# Autodesk Inventor assembly: V4SlapperTower
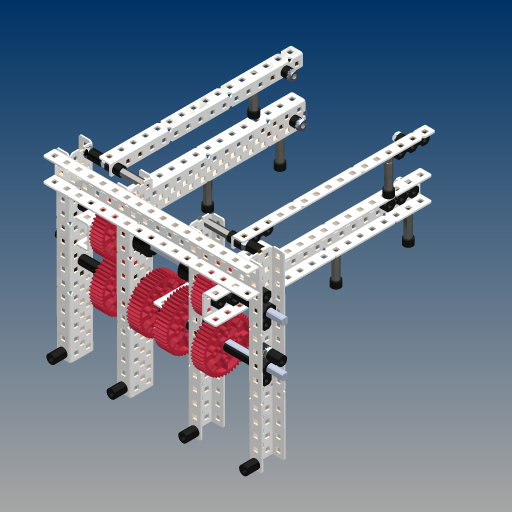
[picture p0: Inventor's stored thumbnail of the model, 512x512]
Saved by Autodesk Inventor 2023 (Build 270158000, 158)
## iProperties
Created: 2024-01-13
Part Number: V4SlapperTower
Document SubType Name: Assembly
Designer: eddie
Author: eddie
## Documents named in this file (30)
- C:\Users\eddie\Documents\81208X-Over-Under-CAD\V4\V4SlapperTower.iam
- C:\Users\eddie\Documents\81208X-Over-Under-CAD\VEX-CAD-Inventor-1.4.0\Structure\C Channel\Aluminum 1x2x1\Alu C 1x2x1x17.ipt
- C:\Users\eddie\Documents\81208X-Over-Under-CAD\VEX-CAD-Inventor-1.4.0\Structure\C Channel\Aluminum 1x2x1\Alu C 1x2x1x15.ipt
- C:\Users\eddie\Documents\81208X-Over-Under-CAD\VEX-CAD-Inventor-1.4.0\Motion\Spacers\Spacer Nylon .375 OD\NSpacer .375 OD x .500.ipt
- C:\Users\eddie\Documents\81208X-Over-Under-CAD\VEX-CAD-Inventor-1.4.0\Motion\Spacers\Spacer Nylon .375 OD.ipt
- C:\Users\eddie\Documents\81208X-Over-Under-CAD\VEX-CAD-Inventor-1.4.0\Motion\Spacers\Spacer Nylon .375 OD\NSpacer .375 OD x .250.ipt
- C:\Users\eddie\Documents\81208X-Over-Under-CAD\VEX-CAD-Inventor-1.4.0\Motion\Shaft HS\HS Bearing Flat.ipt
- C:\Users\eddie\Documents\81208X-Over-Under-CAD\VEX-CAD-Inventor-1.4.0\Motion\Gears\HS Gear\HS 48T Gear, Square.iam
- C:\Users\eddie\Documents\81208X-Over-Under-CAD\VEX-CAD-Inventor-1.4.0\Motion\Gears\HS Gear.iam
- C:\Users\eddie\Documents\81208X-Over-Under-CAD\VEX-CAD-Inventor-1.4.0\Motion\Spacers\Spacer Nylon .375 OD\NSpacer .375 OD x .125.ipt
- C:\Users\eddie\Documents\81208X-Over-Under-CAD\VEX-CAD-Inventor-1.4.0\Structure\Hardware\Nut Keps.ipt
- C:\Users\eddie\Documents\81208X-Over-Under-CAD\VEX-CAD-Inventor-1.4.0\Structure\Standoff\Standoff 1.00.ipt
- C:\Users\eddie\Documents\81208X-Over-Under-CAD\VEX-CAD-Inventor-1.4.0\Structure\Standoff.ipt
- C:\Users\eddie\Documents\81208X-Over-Under-CAD\VEX-CAD-Inventor-1.4.0\Structure\Angle\Aluminum\1x1\Alu Angle 1x1x16.ipt
- C:\Users\eddie\Documents\81208X-Over-Under-CAD\VEX-CAD-Inventor-1.4.0\Motion\Shaft LS\Bearing Flat.ipt
- C:\Users\eddie\Documents\81208X-Over-Under-CAD\VEX-CAD-Inventor-1.4.0\Structure\Hardware\Nut Nylock.ipt
- C:\Users\eddie\Documents\81208X-Over-Under-CAD\VEX-CAD-Inventor-1.4.0\Structure\C Channel\Aluminum 1x2x1\Alu C 1x2x1x18.ipt
- C:\Users\eddie\Documents\81208X-Over-Under-CAD\VEX-CAD-Inventor-1.4.0\Structure\C Channel\Aluminum 1x2x1\Alu C 1x2x1x15_MIR1.ipt
- C:\Users\eddie\Documents\81208X-Over-Under-CAD\VEX-CAD-Inventor-1.4.0\Motion\Shaft HS\HS Bearing Flat_MIR.ipt
- C:\Users\eddie\Documents\81208X-Over-Under-CAD\VEX-CAD-Inventor-1.4.0\Motion\Gears\HS Gear\HS 48T Gear, Square_MIR.iam
- C:\Users\eddie\Documents\81208X-Over-Under-CAD\VEX-CAD-Inventor-1.4.0\Structure\Hardware\Nut Keps_MIR.ipt
- C:\Users\eddie\Documents\81208X-Over-Under-CAD\VEX-CAD-Inventor-1.4.0\Structure\Angle\Aluminum\1x1\Alu Angle 1x1x16_MIR.ipt
- C:\Users\eddie\Documents\81208X-Over-Under-CAD\VEX-CAD-Inventor-1.4.0\Motion\Shaft LS\Bearing Flat_MIR1.ipt
- C:\Users\eddie\Documents\81208X-Over-Under-CAD\VEX-CAD-Inventor-1.4.0\Structure\Hardware\Nut Nylock_MIR.ipt
- C:\Users\eddie\Documents\81208X-Over-Under-CAD\VEX-CAD-Inventor-1.4.0\Structure\C Channel\Aluminum 1x2x1\Alu C 1x2x1x18_MIR.ipt
- C:\Users\eddie\Documents\81208X-Over-Under-CAD\VEX-CAD-Inventor-1.4.0\Structure\C Channel\Aluminum 1x2x1\Alu C 1x2x1x9.ipt
- C:\Users\eddie\Documents\81208X-Over-Under-CAD\VEX-CAD-Inventor-1.4.0\Motion\Shaft HS\Shaft HS\Shaft HS 8.5 in.ipt
- C:\Users\eddie\Documents\81208X-Over-Under-CAD\VEX-CAD-Inventor-1.4.0\Motion\Shaft HS\Shaft HS.ipt
- C:\Users\eddie\Documents\81208X-Over-Under-CAD\VEX-CAD-Inventor-1.4.0\Motion\Shaft HS\HS Shaft Collar.ipt
- C:\Users\eddie\Documents\81208X-Over-Under-CAD\VEX-CAD-Inventor-1.4.0\Structure\Standoff\Standoff .25.ipt
## Components (100 placed, 25 different names)
1. Alu C 1x2x1x15:1 — Insert:8, Insert:9, Insert:24, Insert:25, Insert:36, Insert:75, Insert:76
2. Alu C 1x2x1x15:2 — Insert:7, Insert:13, Insert:17, Insert:28, Insert:31, Insert:74, Insert:77, Insert:84
3. NSpacer .375 OD x .500:1 — Insert:8
4. NSpacer .375 OD x .500:2 — Insert:7
5. NSpacer .375 OD x .500:5 — Insert:9, Insert:11
6. NSpacer .375 OD x .250:7 — Insert:11, Insert:12
7. NSpacer .375 OD x .500:8 — Insert:12
8. HS Bearing Flat:1 — Insert:13, Insert:14
9. NSpacer .375 OD x .250:9 — Insert:14, Insert:15
10. HS 48T Gear, Square:1 [sub-assembly] — Insert:15, Insert:38
11. HS Bearing Flat:2 — Insert:17, Insert:18
12. NSpacer .375 OD x .250:11 — Insert:18, Insert:19
13. HS 48T Gear, Square:2 [sub-assembly] — Insert:19, Insert:20
14. NSpacer .375 OD x .125:12 — Insert:20, Insert:21
15. NSpacer .375 OD x .500:13 — Insert:21, Insert:22
16. NSpacer .375 OD x .500:14 — Insert:22, Insert:23
17. NSpacer .375 OD x .250:15 — Insert:23
18. HS Bearing Flat:3 — Insert:24, Insert:82
19. HS Bearing Flat:4 — Insert:25, Insert:26, Insert:83
20. Nut Keps:1 — Insert:26, Insert:27
21. NSpacer .375 OD x .500:16 — Insert:27
22. NSpacer .375 OD x .250:17 — Insert:28, Insert:29
23. NSpacer .375 OD x .125:18 — Insert:29, Insert:30
24. HS 48T Gear, Square:3 [sub-assembly] — Insert:30
25. Standoff 1.00:1 — Insert:31, Insert:32
26. NSpacer .375 OD x .250:19 — Insert:32, Insert:33
27. Alu Angle 1x1x16:1 — Insert:33, Insert:34, Insert:78, Insert:86, Insert:102, Insert:108
28. Bearing Flat:1 — Insert:34, Insert:35, Insert:78
29. Nut Nylock:1 — Insert:35
30. Nut Keps:2 — Insert:36, Insert:37
31. NSpacer .375 OD x .500:20 — Insert:37
32. Alu C 1x2x1x18:1 — Insert:38, Insert:39, Insert:40, Insert:87, Insert:94, Insert:100, Insert:116
33. HS Bearing Flat:5 — Insert:39, Insert:40
34. Alu C 1x2x1x15_MIR1:1 — Insert:41, Insert:43, Insert:56, Insert:57, Insert:68, Insert:73
35. Alu C 1x2x1x15_MIR1:2 — Insert:42, Insert:46, Insert:49, Insert:60, Insert:63, Insert:85
36. NSpacer .375 OD x .500:21 — Insert:41
37. NSpacer .375 OD x .500:22 — Insert:42
38. NSpacer .375 OD x .500:23 — Insert:43, Insert:44
39. NSpacer .375 OD x .250:24 — Insert:44, Insert:45
40. NSpacer .375 OD x .500:25 — Insert:45
41. HS Bearing Flat_MIR:1 — Insert:46, Insert:47
42. NSpacer .375 OD x .250:26 — Insert:47, Insert:48
43. HS 48T Gear, Square_MIR:1 [sub-assembly] — Insert:48, Insert:70
44. HS Bearing Flat_MIR:2 — Insert:49, Insert:50
45. NSpacer .375 OD x .250:27 — Insert:50, Insert:51
46. HS 48T Gear, Square_MIR:2 [sub-assembly] — Insert:51, Insert:52
47. NSpacer .375 OD x .125:28 — Insert:52, Insert:53
48. NSpacer .375 OD x .500:29 — Insert:53, Insert:54
49. NSpacer .375 OD x .500:30 — Insert:54, Insert:55
50. NSpacer .375 OD x .250:31 — Insert:55
51. HS Bearing Flat_MIR:3 — Insert:56
52. HS Bearing Flat_MIR:4 — Insert:57, Insert:58
53. Nut Keps_MIR:1 — Insert:58, Insert:59
54. NSpacer .375 OD x .500:32 — Insert:59
55. NSpacer .375 OD x .250:33 — Insert:60, Insert:61
56. NSpacer .375 OD x .125:34 — Insert:61, Insert:62
57. HS 48T Gear, Square_MIR:3 [sub-assembly] — Insert:62, Insert:79
58. Standoff 1.00:2 — Insert:63, Insert:64
59. NSpacer .375 OD x .250:35 — Insert:64, Insert:65
60. Alu Angle 1x1x16_MIR:1 — Insert:65, Insert:66, Insert:88, Insert:105, Insert:110
61. Bearing Flat_MIR1:1 — Insert:66, Insert:67
62. Nut Nylock_MIR:1 — Insert:67
63. Nut Keps_MIR:2 — Insert:68, Insert:69
64. NSpacer .375 OD x .500:36 — Insert:69
65. Alu C 1x2x1x18_MIR:1 — Insert:70, Insert:71, Insert:72, Insert:89, Insert:96, Insert:97, Insert:114
66. HS Bearing Flat_MIR:5 — Insert:71, Insert:72
67. Alu C 1x2x1x17:1 — Insert:73, Insert:74, Insert:75, Insert:76, Insert:77
68. Alu C 1x2x1x9:1 — Insert:79, Insert:80
69. NSpacer .375 OD x .500:37 — Insert:80, Insert:81
70. NSpacer .375 OD x .125:38 — Insert:81
71. Shaft HS 8.5 in:1 — Insert:82
72. Shaft HS 8.5 in:2 — Insert:83
73. HS Shaft Collar:1 — Insert:84
74. HS Shaft Collar:2 — Insert:85
75. Bearing Flat:2 — Insert:86
76. Bearing Flat:3 — Insert:87
77. Bearing Flat:4 — Insert:88
78. Bearing Flat:5 — Insert:89
79. Standoff 1.00:5 — Insert:94, Insert:95
80. NSpacer .375 OD x .250:41 — Insert:95
81. Standoff 1.00:6 — Insert:96, Insert:98
82. Standoff 1.00:7 — Insert:97, Insert:99
83. NSpacer .375 OD x .250:42 — Insert:98
84. NSpacer .375 OD x .250:43 — Insert:99
85. Standoff 1.00:8 — Insert:100, Insert:101
86. NSpacer .375 OD x .250:44 — Insert:101
87. Standoff .25:9 — Insert:102, Insert:103
88. Standoff 1.00:10 — Insert:103, Insert:104
89. NSpacer .375 OD x .250:45 — Insert:104
90. Standoff .25:11 — Insert:105, Insert:106
91. Standoff 1.00:12 — Insert:106, Insert:107
92. NSpacer .375 OD x .250:46 — Insert:107
93. NSpacer .375 OD x .250:47 — Insert:108, Insert:109
94. Nut Keps:3 — Insert:109
95. NSpacer .375 OD x .250:48 — Insert:110, Insert:111
96. Nut Keps:4 — Insert:111
97. NSpacer .375 OD x .250:50 — Insert:114, Insert:115
98. Nut Keps:6 — Insert:115
99. NSpacer .375 OD x .250:51 — Insert:116, Insert:117
100. Nut Keps:7 — Insert:117
## Relationships (103: Insert 103)
- Insert:7: Alu C 1x2x1x15:2 ↔ NSpacer .375 OD x .500:2
- Insert:8: Alu C 1x2x1x15:1 ↔ NSpacer .375 OD x .500:1
- Insert:9: Alu C 1x2x1x15:1 ↔ NSpacer .375 OD x .500:5
- Insert:11: NSpacer .375 OD x .500:5 ↔ NSpacer .375 OD x .250:7
- Insert:12: NSpacer .375 OD x .250:7 ↔ NSpacer .375 OD x .500:8
- Insert:13: Alu C 1x2x1x15:2 ↔ HS Bearing Flat:1
- Insert:14: HS Bearing Flat:1 ↔ NSpacer .375 OD x .250:9
- Insert:15: NSpacer .375 OD x .250:9 ↔ HS 48T Gear, Square:1
- Insert:17: Alu C 1x2x1x15:2 ↔ HS Bearing Flat:2
- Insert:18: HS Bearing Flat:2 ↔ NSpacer .375 OD x .250:11
- Insert:19: NSpacer .375 OD x .250:11 ↔ HS 48T Gear, Square:2
- Insert:20: HS 48T Gear, Square:2 ↔ NSpacer .375 OD x .125:12
- Insert:21: NSpacer .375 OD x .125:12 ↔ NSpacer .375 OD x .500:13
- Insert:22: NSpacer .375 OD x .500:13 ↔ NSpacer .375 OD x .500:14
- Insert:23: NSpacer .375 OD x .500:14 ↔ NSpacer .375 OD x .250:15
- Insert:24: Alu C 1x2x1x15:1 ↔ HS Bearing Flat:3
- Insert:25: Alu C 1x2x1x15:1 ↔ HS Bearing Flat:4
- Insert:26: HS Bearing Flat:4 ↔ Nut Keps:1
- Insert:27: Nut Keps:1 ↔ NSpacer .375 OD x .500:16
- Insert:28: Alu C 1x2x1x15:2 ↔ NSpacer .375 OD x .250:17
- Insert:29: NSpacer .375 OD x .250:17 ↔ NSpacer .375 OD x .125:18
- Insert:30: NSpacer .375 OD x .125:18 ↔ HS 48T Gear, Square:3
- Insert:31: Alu C 1x2x1x15:2 ↔ Standoff 1.00:1
- Insert:32: Standoff 1.00:1 ↔ NSpacer .375 OD x .250:19
- Insert:33: NSpacer .375 OD x .250:19 ↔ Alu Angle 1x1x16:1
- Insert:34: Alu Angle 1x1x16:1 ↔ Bearing Flat:1
- Insert:35: Bearing Flat:1 ↔ Nut Nylock:1
- Insert:36: Alu C 1x2x1x15:1 ↔ Nut Keps:2
- Insert:37: Nut Keps:2 ↔ NSpacer .375 OD x .500:20
- Insert:38: HS 48T Gear, Square:1 ↔ Alu C 1x2x1x18:1
- Insert:39: Alu C 1x2x1x18:1 ↔ HS Bearing Flat:5
- Insert:40: Alu C 1x2x1x18:1 ↔ HS Bearing Flat:5
- Insert:41: Alu C 1x2x1x15_MIR1:1 ↔ NSpacer .375 OD x .500:21
- Insert:42: Alu C 1x2x1x15_MIR1:2 ↔ NSpacer .375 OD x .500:22
- Insert:43: Alu C 1x2x1x15_MIR1:1 ↔ NSpacer .375 OD x .500:23
- Insert:44: NSpacer .375 OD x .500:23 ↔ NSpacer .375 OD x .250:24
- Insert:45: NSpacer .375 OD x .250:24 ↔ NSpacer .375 OD x .500:25
- Insert:46: Alu C 1x2x1x15_MIR1:2 ↔ HS Bearing Flat_MIR:1
- Insert:47: HS Bearing Flat_MIR:1 ↔ NSpacer .375 OD x .250:26
- Insert:48: NSpacer .375 OD x .250:26 ↔ HS 48T Gear, Square_MIR:1
- Insert:49: Alu C 1x2x1x15_MIR1:2 ↔ HS Bearing Flat_MIR:2
- Insert:50: HS Bearing Flat_MIR:2 ↔ NSpacer .375 OD x .250:27
- Insert:51: NSpacer .375 OD x .250:27 ↔ HS 48T Gear, Square_MIR:2
- Insert:52: HS 48T Gear, Square_MIR:2 ↔ NSpacer .375 OD x .125:28
- Insert:53: NSpacer .375 OD x .125:28 ↔ NSpacer .375 OD x .500:29
- Insert:54: NSpacer .375 OD x .500:29 ↔ NSpacer .375 OD x .500:30
- Insert:55: NSpacer .375 OD x .500:30 ↔ NSpacer .375 OD x .250:31
- Insert:56: Alu C 1x2x1x15_MIR1:1 ↔ HS Bearing Flat_MIR:3
- Insert:57: Alu C 1x2x1x15_MIR1:1 ↔ HS Bearing Flat_MIR:4
- Insert:58: HS Bearing Flat_MIR:4 ↔ Nut Keps_MIR:1
- Insert:59: Nut Keps_MIR:1 ↔ NSpacer .375 OD x .500:32
- Insert:60: Alu C 1x2x1x15_MIR1:2 ↔ NSpacer .375 OD x .250:33
- Insert:61: NSpacer .375 OD x .250:33 ↔ NSpacer .375 OD x .125:34
- Insert:62: NSpacer .375 OD x .125:34 ↔ HS 48T Gear, Square_MIR:3
- Insert:63: Alu C 1x2x1x15_MIR1:2 ↔ Standoff 1.00:2
- Insert:64: Standoff 1.00:2 ↔ NSpacer .375 OD x .250:35
- Insert:65: NSpacer .375 OD x .250:35 ↔ Alu Angle 1x1x16_MIR:1
- Insert:66: Alu Angle 1x1x16_MIR:1 ↔ Bearing Flat_MIR1:1
- Insert:67: Bearing Flat_MIR1:1 ↔ Nut Nylock_MIR:1
- Insert:68: Alu C 1x2x1x15_MIR1:1 ↔ Nut Keps_MIR:2
- Insert:69: Nut Keps_MIR:2 ↔ NSpacer .375 OD x .500:36
- Insert:70: HS 48T Gear, Square_MIR:1 ↔ Alu C 1x2x1x18_MIR:1
- Insert:71: Alu C 1x2x1x18_MIR:1 ↔ HS Bearing Flat_MIR:5
- Insert:72: Alu C 1x2x1x18_MIR:1 ↔ HS Bearing Flat_MIR:5
- Insert:73: Alu C 1x2x1x15_MIR1:1 ↔ Alu C 1x2x1x17:1
- Insert:74: Alu C 1x2x1x15:2 ↔ Alu C 1x2x1x17:1
- Insert:75: Alu C 1x2x1x15:1 ↔ Alu C 1x2x1x17:1
- Insert:76: Alu C 1x2x1x15:1 ↔ Alu C 1x2x1x17:1
- Insert:77: Alu C 1x2x1x15:2 ↔ Alu C 1x2x1x17:1
- Insert:78: Alu Angle 1x1x16:1 ↔ Bearing Flat:1
- Insert:79: HS 48T Gear, Square_MIR:3 ↔ Alu C 1x2x1x9:1
- Insert:80: Alu C 1x2x1x9:1 ↔ NSpacer .375 OD x .500:37
- Insert:81: NSpacer .375 OD x .500:37 ↔ NSpacer .375 OD x .125:38
- Insert:82: HS Bearing Flat:3 ↔ Shaft HS 8.5 in:1
- Insert:83: HS Bearing Flat:4 ↔ Shaft HS 8.5 in:2
- Insert:84: Alu C 1x2x1x15:2 ↔ HS Shaft Collar:1
- Insert:85: Alu C 1x2x1x15_MIR1:2 ↔ HS Shaft Collar:2
- Insert:86: Alu Angle 1x1x16:1 ↔ Bearing Flat:2
- Insert:87: Alu C 1x2x1x18:1 ↔ Bearing Flat:3
- Insert:88: Alu Angle 1x1x16_MIR:1 ↔ Bearing Flat:4
- Insert:89: Alu C 1x2x1x18_MIR:1 ↔ Bearing Flat:5
- Insert:94: Alu C 1x2x1x18:1 ↔ Standoff 1.00:5
- Insert:95: Standoff 1.00:5 ↔ NSpacer .375 OD x .250:41
- Insert:96: Alu C 1x2x1x18_MIR:1 ↔ Standoff 1.00:6
- Insert:97: Alu C 1x2x1x18_MIR:1 ↔ Standoff 1.00:7
- Insert:98: Standoff 1.00:6 ↔ NSpacer .375 OD x .250:42
- Insert:99: Standoff 1.00:7 ↔ NSpacer .375 OD x .250:43
- Insert:100: Alu C 1x2x1x18:1 ↔ Standoff 1.00:8
- Insert:101: Standoff 1.00:8 ↔ NSpacer .375 OD x .250:44
- Insert:102: Alu Angle 1x1x16:1 ↔ Standoff .25:9
- Insert:103: Standoff .25:9 ↔ Standoff 1.00:10
- Insert:104: Standoff 1.00:10 ↔ NSpacer .375 OD x .250:45
- Insert:105: Alu Angle 1x1x16_MIR:1 ↔ Standoff .25:11
- Insert:106: Standoff .25:11 ↔ Standoff 1.00:12
- Insert:107: Standoff 1.00:12 ↔ NSpacer .375 OD x .250:46
- Insert:108: Alu Angle 1x1x16:1 ↔ NSpacer .375 OD x .250:47
- Insert:109: NSpacer .375 OD x .250:47 ↔ Nut Keps:3
- Insert:110: Alu Angle 1x1x16_MIR:1 ↔ NSpacer .375 OD x .250:48
- Insert:111: NSpacer .375 OD x .250:48 ↔ Nut Keps:4
- Insert:114: Alu C 1x2x1x18_MIR:1 ↔ NSpacer .375 OD x .250:50
- Insert:115: NSpacer .375 OD x .250:50 ↔ Nut Keps:6
- Insert:116: Alu C 1x2x1x18:1 ↔ NSpacer .375 OD x .250:51
- Insert:117: NSpacer .375 OD x .250:51 ↔ Nut Keps:7
